# Autodesk Inventor assembly: захват
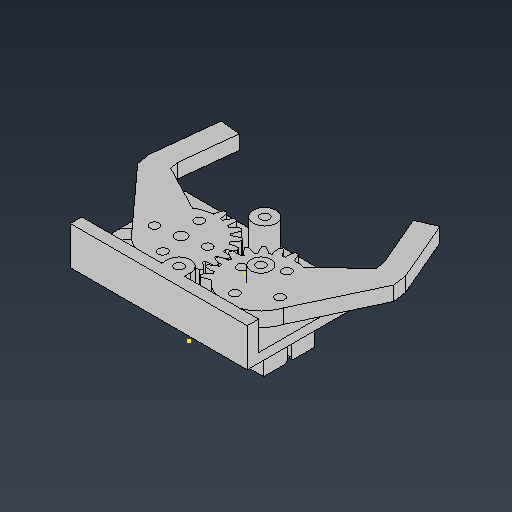
[picture p0: Inventor's stored thumbnail of the model, 512x512]
Saved by Autodesk Inventor 2025 (Build 290162000, 162)
## iProperties
Created: 2025-02-17
Part Number: захват
Document SubType Name: Assembly
Designer: GameHD
Author: GameHD
## Documents named in this file (5)
- C:\Users\GameHD\Desktop\Phantom 16950\захват.iam
- C:\Users\GameHD\Desktop\phantom 16950\ПЕРЕДНИЙ ЗАХВАТ.ipt
- C:\Users\GameHD\Desktop\phantom 16950\писюн 2.ipt
- C:\Users\GameHD\Desktop\phantom 16950\писюн.ipt
- C:\Users\GameHD\Desktop\phantom 16950\2000-0025-0002\2000-0025-0002_MIR4_MIR1_MIR.ipt
## Components (4 placed, 4 different names)
1. ПЕРЕДНИЙ ЗАХВАТ:1 — Совмещение:1, Совмещение:2, Совмещение:3, Совмещение:4, Совмещение:5, Совмещение:6
2. писюн 2:1 — Совмещение:2, Совмещение:4
3. писюн:1 — Совмещение:1, Совмещение:3
4. 2000-0025-0002_MIR4_MIR1_MIR:1 — Совмещение:5, Совмещение:6
## Relationships (6: Mate 6)
- Совмещение:1 [Mate]: ПЕРЕДНИЙ ЗАХВАТ:1 ↔ писюн:1
- Совмещение:2 [Mate]: ПЕРЕДНИЙ ЗАХВАТ:1 ↔ писюн 2:1
- Совмещение:3 [Mate]: ПЕРЕДНИЙ ЗАХВАТ:1 ↔ писюн:1
- Совмещение:4 [Mate]: ПЕРЕДНИЙ ЗАХВАТ:1 ↔ писюн 2:1
- Совмещение:5 [Mate]: ПЕРЕДНИЙ ЗАХВАТ:1 ↔ 2000-0025-0002_MIR4_MIR1_MIR:1
- Совмещение:6 [Mate]: ПЕРЕДНИЙ ЗАХВАТ:1 ↔ 2000-0025-0002_MIR4_MIR1_MIR:1
